# Autodesk Inventor assembly: Gear Set With Spacer
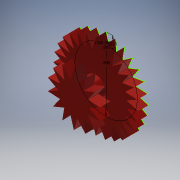
[picture p0: Inventor's stored thumbnail of the model, 180x180]
Saved by Autodesk Inventor 2018 (Build 220112000, 112)
## iProperties
Created: 2018-09-18
Part Number: Gear Set With Spacer
Document SubType Name: Assembly
Designer: User
Author: User
## Documents named in this file (4)
- D:\Gear Set With Spacer.iam
- D:\Big Gear Phone Case Mech.ipt
- D:\Small Gear Phone Case Mech.ipt
- D:\Spacer.ipt
## Components (3 placed, 3 different names)
1. Big Gear Phone Case Mech:1 — Insert:1
2. Spacer:1 — Insert:1, Insert:2
3. Small Gear Phone Case Mech:1 — Insert:2
## Relationships (2: Insert 2)
- Insert:1: Big Gear Phone Case Mech:1 ↔ Spacer:1
- Insert:2: Spacer:1 ↔ Small Gear Phone Case Mech:1
